# Autodesk Inventor assembly: wheel_ass_s1
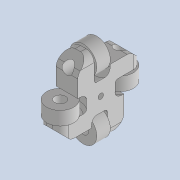
[picture p0: Inventor's stored thumbnail of the model, 180x180]
Saved by Autodesk Inventor 2020 (Build 240168000, 168)
## iProperties
Created: 2021-12-22
Part Number: wheel_ass_s1
Document SubType Name: Assembly
Designer: Shuang Peng
Author: Shuang Peng
## Documents named in this file (3)
- D:\projects-3\soft module robot\hardware\diff module 3\wheel_ass_s1.iam
- D:\projects-3\soft module robot\hardware\diff module 3\bearing_2_5_2.5.ipt
- D:\projects-3\soft module robot\hardware\diff module 3\wheel_t1.ipt
## Components (5 placed, 2 different names)
1. bearing_2_5_2.5:1 — Flush:1, Insert:1
2. wheel_t1:1 — Flush:1, Insert:1, Insert:2, Insert:3, Insert:4
3. bearing_2_5_2.5:2 — Insert:2
4. bearing_2_5_2.5:3 — Insert:3
5. bearing_2_5_2.5:4 — Insert:4
## Relationships (5: Insert 4, Flush 1)
- Flush:1: bearing_2_5_2.5:1 ↔ wheel_t1:1
- Insert:1: bearing_2_5_2.5:1 ↔ wheel_t1:1
- Insert:2: wheel_t1:1 ↔ bearing_2_5_2.5:2
- Insert:3: wheel_t1:1 ↔ bearing_2_5_2.5:3
- Insert:4: wheel_t1:1 ↔ bearing_2_5_2.5:4
